# Autodesk Inventor assembly: u_k_Hoehenverstellung_Seiten
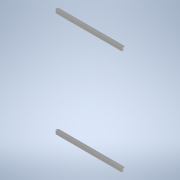
[picture p0: Inventor's stored thumbnail of the model, 180x180]
Saved by Autodesk Inventor 2020.3 (Build 243373000, 373)
## iProperties
Created: 2020-10-04
Part Number: u_k_Hoehenverstellung_Seiten
Document SubType Name: Assembly
Designer: Mara
Author: Mara
## Documents named in this file (2)
- C:\Users\Mara\Masterarbeit_CAD\Rampe\u_k_Hoehenverstellung_Seiten.iam
- C:\Users\Mara\Masterarbeit_CAD\Rampe\u_k_Hoehenverstellung_Seiten.ipt
## Components (2 placed, 1 different names)
1. u_k_Hoehenverstellung_Seiten:1 — Mate:1, Flush:1, Tangent:1
2. u_k_Hoehenverstellung_Seiten:2 — Mate:1, Flush:1, Tangent:1
## Relationships (3: Mate 1, Flush 1, Tangent 1)
- Mate:1 (664 mm): u_k_Hoehenverstellung_Seiten:1 ↔ u_k_Hoehenverstellung_Seiten:2
- Flush:1: u_k_Hoehenverstellung_Seiten:1 ↔ u_k_Hoehenverstellung_Seiten:2
- Tangent:1: u_k_Hoehenverstellung_Seiten:1 ↔ u_k_Hoehenverstellung_Seiten:2
